# Autodesk Inventor assembly: Assembly_Cube_Kinematic_Mirrormount_30x30_45_Asromedia_Partiallytransparent_30x40x1mmv3
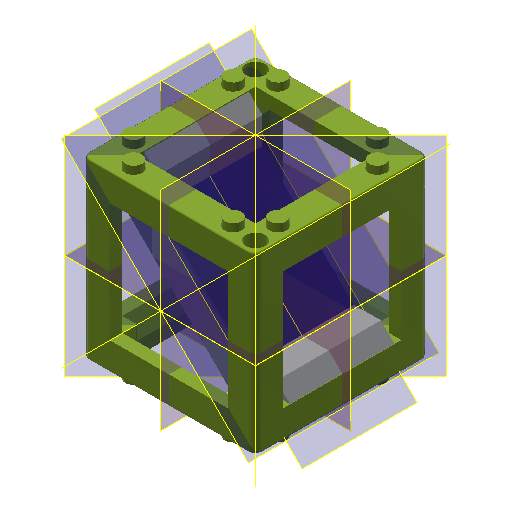
[picture p0: Inventor's stored thumbnail of the model, 512x512]
Saved by Autodesk Inventor 2022 (Build 260153000, 153)
## iProperties
Created: 2020-03-27
Part Number: Assembly_Cube_Kinematic_Mirrormount_30x30_45_Asromedia_Partiallytransparent_30x40x1mmv3
Document SubType Name: Assembly
Designer: B
Mass: 27.8603 g
Surface Area: 235.464 cm^2
Volume: 27.8603 cm^3
Density: 1 g/cm^3
Author: B
## Documents named in this file (4)
- C:\Users\diederichbenedict\Dropbox\Dokumente\Promotion\PROJECTS\openUC2-CAD\INVENTOR\Assembly_Cube_Beamsplitter_Astromedia_Partiallytransparent_30x40x1mmv3.iam
- C:\Users\diederichbenedict\Dropbox\Dokumente\Promotion\PROJECTS\openUC2-CAD\INVENTOR\Assembly_Cube_empty_IM_v3.iam
- C:\Users\diederichbenedict\Dropbox\Dokumente\Promotion\PROJECTS\openUC2-CAD\INVENTOR\00_Astromedia_FronSurfaceMirror_40x30mmx1mm.ipt
- C:\Users\diederichbenedict\Dropbox\Dokumente\Promotion\PROJECTS\openUC2-CAD\INVENTOR\20_Cube_Insert_Mirror_Holder_wLogo_PartiallyTransparent_Astromedia_30x40x1_v3.ipt
## Components (3 placed, 3 different names)
1. 20_Cube_Insert_Mirror_Holder_wLogo_PartiallyTransparent_Astromedia_30x40x1_v3:1 — Passend:1, Fluchtend:1, Passend:3, Passend:4
2. Assembly_Cube_empty_IM_v3:1 [sub-assembly] — Passend:1, Fluchtend:1, Passend:2
3. 00_Astromedia_FronSurfaceMirror_40x30mmx1mm:1 — Passend:2, Passend:3, Passend:4
## Relationships (5: Mate 4, Flush 1)
- Passend:1 [Mate]: 20_Cube_Insert_Mirror_Holder_wLogo_PartiallyTransparent_Astromedia_30x40x1_v3:1 ↔ Assembly_Cube_empty_IM_v3:1
- Fluchtend:1 [Flush]: 20_Cube_Insert_Mirror_Holder_wLogo_PartiallyTransparent_Astromedia_30x40x1_v3:1 ↔ Assembly_Cube_empty_IM_v3:1
- Passend:2 [Mate]: Assembly_Cube_empty_IM_v3:1 ↔ 00_Astromedia_FronSurfaceMirror_40x30mmx1mm:1
- Passend:3 [Mate]: 20_Cube_Insert_Mirror_Holder_wLogo_PartiallyTransparent_Astromedia_30x40x1_v3:1 ↔ 00_Astromedia_FronSurfaceMirror_40x30mmx1mm:1
- Passend:4 [Mate]: 20_Cube_Insert_Mirror_Holder_wLogo_PartiallyTransparent_Astromedia_30x40x1_v3:1 ↔ 00_Astromedia_FronSurfaceMirror_40x30mmx1mm:1
